# Autodesk Inventor assembly: CT2x2
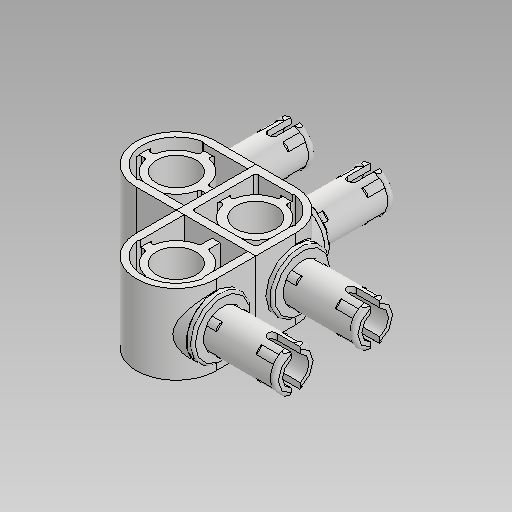
[picture p0: Inventor's stored thumbnail of the model, 512x512]
Saved by Autodesk Inventor 2020 (Build 240168000, 168)
## iProperties
Created: 2019-05-05
Part Number: CT2x2
Document SubType Name: Assembly
Designer: Varga Daniel
Author: Varga Daniel
## Documents named in this file (5)
- C:\!_Dani\!_cloud\OneDrive\!_munka\Revolution\StructuralParts\Connector Boxes\Connector Triangle\CT2x2.iam
- C:\!_Dani\!_cloud\OneDrive\!_munka\Revolution\StructuralParts\Connector Boxes\Connector_triangle_corner.ipt
- C:\!_Dani\!_cloud\OneDrive\!_munka\Revolution\StructuralParts\Beams\beam_single_end_part.ipt
- C:\!_Dani\!_cloud\OneDrive\!_munka\Revolution\StructuralParts\Connector pins\CP1_base\CP1_base-one_side_anti_skid.ipt
- C:\!_Dani\!_cloud\OneDrive\!_munka\Revolution\StructuralParts\Connector pins\CP1_base.ipt
## Components (7 placed, 3 different names)
1. Connector_triangle_corner:1 — Mate:1, Mate:2, Flush:1, Flush:2, Flush:3, Flush:4, Mate:4, Mate:5, Mate:7, Flush:5, Flush:6, Mate:8
2. beam_single_end_part:1 — Mate:1, Flush:2, Flush:3, Mate:3, Flush:9, Mate:9
3. beam_single_end_part:2 — Mate:2, Flush:1, Flush:4, Mate:6, Flush:7, Flush:8
4. CP1_base-one_side_anti_skid:1 — Mate:3, Flush:9, Mate:9
5. CP1_base-one_side_anti_skid:2 — Mate:4, Mate:7, Flush:5
6. CP1_base-one_side_anti_skid:3 — Mate:5, Flush:6, Mate:8
7. CP1_base-one_side_anti_skid:4 — Mate:6, Flush:7, Flush:8
## Relationships (18: Mate 9, Flush 9)
- Mate:1: Connector_triangle_corner:1 ↔ beam_single_end_part:1
- Mate:2: Connector_triangle_corner:1 ↔ beam_single_end_part:2
- Flush:1: Connector_triangle_corner:1 ↔ beam_single_end_part:2
- Flush:2: Connector_triangle_corner:1 ↔ beam_single_end_part:1
- Flush:3: Connector_triangle_corner:1 ↔ beam_single_end_part:1
- Flush:4: Connector_triangle_corner:1 ↔ beam_single_end_part:2
- Mate:3: beam_single_end_part:1 ↔ CP1_base-one_side_anti_skid:1
- Mate:4: Connector_triangle_corner:1 ↔ CP1_base-one_side_anti_skid:2
- Mate:5: Connector_triangle_corner:1 ↔ CP1_base-one_side_anti_skid:3
- Mate:6: beam_single_end_part:2 ↔ CP1_base-one_side_anti_skid:4
- Mate:7: Connector_triangle_corner:1 ↔ CP1_base-one_side_anti_skid:2
- Flush:5: Connector_triangle_corner:1 ↔ CP1_base-one_side_anti_skid:2
- Flush:6: Connector_triangle_corner:1 ↔ CP1_base-one_side_anti_skid:3
- Mate:8: Connector_triangle_corner:1 ↔ CP1_base-one_side_anti_skid:3
- Flush:7: beam_single_end_part:2 ↔ CP1_base-one_side_anti_skid:4
- Flush:8: beam_single_end_part:2 ↔ CP1_base-one_side_anti_skid:4
- Flush:9: beam_single_end_part:1 ↔ CP1_base-one_side_anti_skid:1
- Mate:9: beam_single_end_part:1 ↔ CP1_base-one_side_anti_skid:1
